# Autodesk Inventor assembly: CE-8.2.1
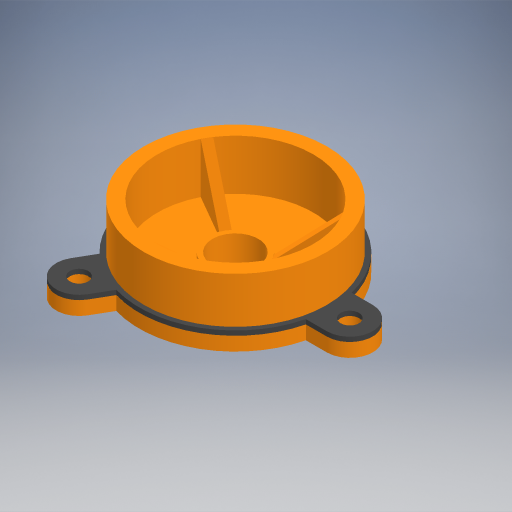
[picture p0: Inventor's stored thumbnail of the model, 512x512]
Saved by Autodesk Inventor 2024 (Build 280153000, 153)
## iProperties
Created: 2024-03-07
Part Number: CE-8.2.1
Document SubType Name: Assembly
Designer: Alex
Author: Alex
## Documents named in this file (4)
- C:\Shared\alex-bartella-schoolwork\4z03\Week 8\CE-8.2.1.iam
- C:\Shared\alex-bartella-schoolwork\4z03\Week 8\CE-2.1.4_1.ipt
- C:\Shared\alex-bartella-schoolwork\4z03\Week 8\CE-2.1.4.ipt
- C:\Shared\alex-bartella-schoolwork\4z03\Week 8\CE-8.2.1-01-001.ipt
## Components (2 placed, 2 different names)
1. CE-2.1.4_1:1 — Flush:1
2. CE-8.2.1-01-001:1 — Flush:1
## Relationships (1: Flush 1)
- Flush:1: CE-2.1.4_1:1 ↔ CE-8.2.1-01-001:1
